# Autodesk Inventor assembly: Assembly1
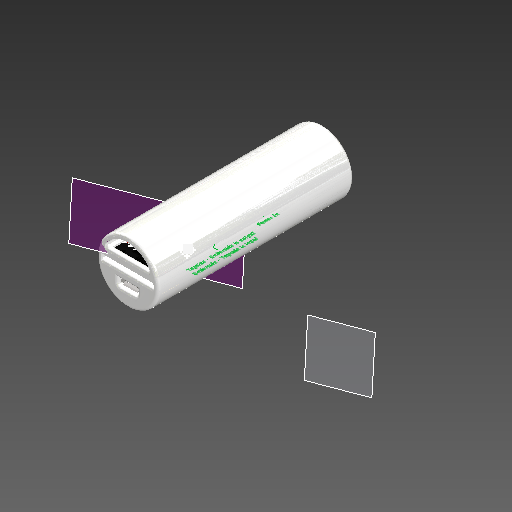
[picture p0: Inventor's stored thumbnail of the model, 512x512]
Saved by Autodesk Inventor 2023.1 (Build 271208000, 208)
## iProperties
Created: 2022-02-20
Part Number: Assembly1
Document SubType Name: Assembly
Designer: Michael Lacey
Mass: 52.8368 g
Surface Area: 254.425 cm^2
Volume: 21.2696 cm^3
Density: 2.48415 g/cm^3
Author: Michael Lacey
## Documents named in this file (8)
- C:\Users\foams\OneDrive\3D Objects\Light Saber\All Files Compiled\CAD\Assembly1.iam
- C:\Users\foams\OneDrive\3D Objects\Light Saber\All Files Compiled\Librarys\arduino-nano-33-iot-1.snapshot.3\Arduino Nano 33 IoT.iam
- C:\Users\foams\OneDrive\3D Objects\Light Saber\All Files Compiled\CAD\Proto-Board.ipt
- C:\Users\foams\OneDrive\3D Objects\Light Saber\All Files Compiled\Librarys\User Library-integrated circuit DIP14\User Library-integrated circuit DIP14.ipt
- C:\Users\foams\OneDrive\3D Objects\Light Saber\All Files Compiled\CAD\TO-220 3pins long V1.ipt
- C:\Users\foams\OneDrive\3D Objects\Light Saber\All Files Compiled\CAD\Electronics Housing.ipt
- C:\Users\foams\OneDrive\3D Objects\Light Saber\All Files Compiled\CAD\3350 RGB button.ipt
- C:\Users\foams\OneDrive\3D Objects\Light Saber\All Files Compiled\Assembly1\AIP\Cable and Harness\Assembly1.Harness1.iam
## Components (7 placed, 7 different names)
1. Arduino Nano 33 IoT:1 [sub-assembly] — Mate:3, Flush:5, Flush:6
2. Proto-Board:1 — Mate:2, Flush:3, Mate:3, Flush:5, Flush:6, Mate:6, Mate:8, Flush:9, Flush:10, Mate:10, Mate:11, Mate:15, Mate:16
3. User Library-integrated circuit DIP14:1 — Mate:2, Flush:3
4. TO-220 3pins long V1:1 — Mate:8, Flush:9, Flush:10
5. Electronics Housing:1 — Mate:6, Mate:10, Mate:11, Mate:12
6. 3350 RGB button:1 — Mate:12, Mate:13, Mate:14
7. Wiring [sub-assembly]
## Relationships (17: Mate 12, Flush 5)
- Mate:2 (1.27 mm): Proto-Board:1 ↔ User Library-integrated circuit DIP14:1
- Flush:3 (6.096 mm): Proto-Board:1 ↔ User Library-integrated circuit DIP14:1
- Mate:3 (5.08 mm): Arduino Nano 33 IoT:1 ↔ Proto-Board:1
- Flush:5: Arduino Nano 33 IoT:1 ↔ Proto-Board:1
- Flush:6 (1.1049 mm): Arduino Nano 33 IoT:1 ↔ Proto-Board:1
- Mate:6: Proto-Board:1 ↔ Electronics Housing:1
- Mate:8: Proto-Board:1 ↔ TO-220 3pins long V1:1
- Flush:9 (2.9972 mm): Proto-Board:1 ↔ TO-220 3pins long V1:1
- Flush:10 (-25.6286 mm): Proto-Board:1 ↔ TO-220 3pins long V1:1
- Mate:10: Proto-Board:1 ↔ Electronics Housing:1
- Mate:11: Proto-Board:1 ↔ Electronics Housing:1
- Mate:12: Electronics Housing:1 ↔ 3350 RGB button:1
- Mate:13: 3350 RGB button:1
- Mate:14: 3350 RGB button:1
- Mate:15: Proto-Board:1
- Mate:16: Proto-Board:1
- Mate:17
